# Autodesk Inventor assembly: cover3
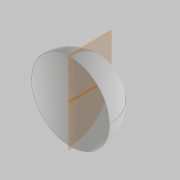
[picture p0: Inventor's stored thumbnail of the model, 180x180]
Saved by Autodesk Inventor 2021 (Build 250183000, 183)
## iProperties
Created: 2021-06-01
Part Number: cover3
Document SubType Name: Assembly
Designer: Watchdog
Author: Watchdog
## Documents named in this file (3)
- C:\Users\Watchdog\OneDrive - Flinders\Advn Mech Design Shared\6_Development\2_Design\inventor\cover\cover3.iam
- C:\Users\Watchdog\OneDrive - Flinders\Advn Mech Design Shared\6_Development\2_Design\inventor\cover\cover2_end.ipt
- C:\Users\Watchdog\OneDrive - Flinders\Advn Mech Design Shared\6_Development\2_Design\inventor\cover\cover2_end_small.ipt
## Components (2 placed, 2 different names)
1. cover2_end:1 — Flush:1, Flush:2, Flush:3, Mate:1, Mate:2
2. cover2_end_small:1 — Flush:2, Mate:2
## Relationships (5: Flush 3, Mate 2)
- Flush:1: cover2_end:1
- Flush:2: cover2_end:1 ↔ cover2_end_small:1
- Flush:3: cover2_end:1
- Mate:1: cover2_end:1
- Mate:2: cover2_end:1 ↔ cover2_end_small:1
